# Autodesk Inventor assembly: phone turning
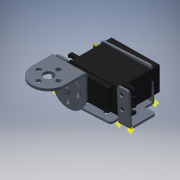
[picture p0: Inventor's stored thumbnail of the model, 180x180]
Saved by Autodesk Inventor 2017 (Build 210142000, 142)
## iProperties
Created: 2017-06-15
Part Number: phone turning
Document SubType Name: Assembly
Designer: slong
Author: slong
## Documents named in this file (4)
- C:\Users\slong\Desktop\ftc robot\phone turning.iam
- C:\Users\slong\Desktop\ftc robot\extracted\tetrix_739060_2012.ipt
- C:\Users\slong\Desktop\ftc robot\extracted\tetrix_739197_2012.iam
- C:\Users\slong\Desktop\ftc robot\extracted\tetrix_739062_2012.ipt
## Components (3 placed, 3 different names)
1. tetrix_739060_2012:1 — Mate:1, Mate:2
2. tetrix_739062_2012:1 — Mate:3, Mate:4
3. tetrix_739197_2012:1 [sub-assembly] — Mate:1, Mate:2, Mate:3, Mate:4
## Relationships (4: Mate 4)
- Mate:1: tetrix_739060_2012:1 ↔ tetrix_739197_2012:1
- Mate:2 (2.54 mm): tetrix_739060_2012:1 ↔ tetrix_739197_2012:1
- Mate:3: tetrix_739062_2012:1 ↔ tetrix_739197_2012:1
- Mate:4: tetrix_739062_2012:1 ↔ tetrix_739197_2012:1
